# Autodesk Inventor assembly: WireBarrelComponent_B
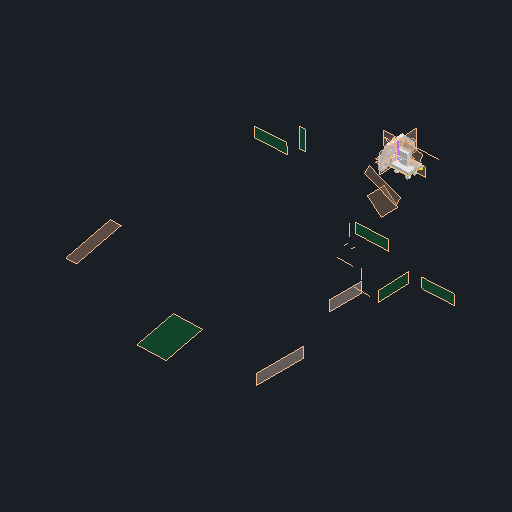
[picture p0: Inventor's stored thumbnail of the model, 512x512]
Saved by Autodesk Inventor 2024.1 (Build 281209000, 209)
## iProperties
Created: 2023-08-17
Part Number: WireBarrelComponent_B
Document SubType Name: Assembly
Designer: Eleanor
Author: Eleanor
## Documents named in this file (4)
- C:\Users\Eleanor\Documents\Inventor\4.5mm ERS\WireBarrelComponent_B.iam
- C:\Users\Eleanor\Documents\Inventor\4.5mm ERS\WireSlottedHoles.iam
- C:\Users\Eleanor\Documents\Inventor\4.5mm ERS\MirrorBaseplate.ipt
- C:\Users\Eleanor\Documents\Inventor\4.5mm ERS\InjectorSystem.ipt
## Components (3 placed, 3 different names)
1. WireSlottedHoles:1 [sub-assembly] — Mate:16, Mate:17, Angle:4, Mate:21, Mate:25, Mate:28, Mate:29, Angle:6, Mate:31, Mate:34
2. MirrorBaseplate:1 — Mate:29, Mate:30, Angle:5, Symmetry:1, Mate:33, Angle:8, Symmetry:3, Mate:35
3. InjectorSystem:1 — Mate:32, Angle:7, Symmetry:2, Mate:34, Mate:35, Mate:37, Mate:38, Mate:40
## Relationships (30: Mate 21, Angle 5, Symmetry 3, Flush 1)
- Mate:7
- Mate:14
- Mate:16: WireSlottedHoles:1
- Mate:17: WireSlottedHoles:1
- Mate:20
- Angle:4 (90 deg): WireSlottedHoles:1
- Mate:21: WireSlottedHoles:1
- Mate:25: WireSlottedHoles:1
- Mate:28: WireSlottedHoles:1
- Mate:29: WireSlottedHoles:1 ↔ MirrorBaseplate:1
- Mate:30: MirrorBaseplate:1
- Angle:5 (0 deg): MirrorBaseplate:1
- Symmetry:1: MirrorBaseplate:1
- Angle:6 (270 deg): WireSlottedHoles:1
- Mate:31: WireSlottedHoles:1
- Mate:32: InjectorSystem:1
- Angle:7 (0 deg): InjectorSystem:1
- Symmetry:2: InjectorSystem:1
- Mate:33: MirrorBaseplate:1
- Angle:8 (0 deg): MirrorBaseplate:1
- Symmetry:3: MirrorBaseplate:1
- Mate:34: WireSlottedHoles:1 ↔ InjectorSystem:1
- Mate:35: MirrorBaseplate:1 ↔ InjectorSystem:1
- Mate:36
- Flush:1
- Mate:37: InjectorSystem:1
- Mate:38: InjectorSystem:1
- Mate:39
- Mate:40: InjectorSystem:1
- Mate:41
